# Autodesk Inventor assembly: DarkCeilingSubassembly
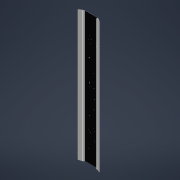
[picture p0: Inventor's stored thumbnail of the model, 180x180]
Saved by Autodesk Inventor 2021 (Build 250183000, 183)
## iProperties
Created: 2021-01-31
Part Number: DarkCeilingSubassembly
Document SubType Name: Assembly
Designer: argon
Author: argon
## Documents named in this file (5)
- C:\Users\argon\OneDrive\Documents\GrabCAD\EngOne Maroons\Ceiling Subassembly\DarkCeilingSubassembly.iam
- C:\Users\argon\OneDrive\Documents\GrabCAD\EngOne Maroons\Ceiling Subassembly\CeilingPanel.ipt
- C:\Users\argon\OneDrive\Documents\GrabCAD\EngOne Maroons\Ceiling Subassembly\StarBackdropPanel.ipt
- C:\Users\argon\OneDrive\Documents\GrabCAD\EngOne Maroons\Ceiling Subassembly\DarkSkyPanel.ipt
- C:\Users\argon\OneDrive\Documents\GrabCAD\EngOne Maroons\Ceiling Subassembly\CeilingLight.ipt
## Components (5 placed, 4 different names)
1. CeilingPanel:1 — Mate:1, Flush:1, Mate:2, Mate:4, Mate:5, Flush:3, Mate:6, Flush:4
2. StarBackdropPanel:1 — Mate:1, Flush:1, Mate:2, Mate:3, Flush:2
3. DarkSkyPanel:1 — Mate:3, Mate:4, Flush:2
4. CeilingLight:1 — Mate:5, Flush:3
5. CeilingLight:2 — Mate:6, Flush:4
## Relationships (10: Mate 6, Flush 4)
- Mate:1: CeilingPanel:1 ↔ StarBackdropPanel:1
- Flush:1: CeilingPanel:1 ↔ StarBackdropPanel:1
- Mate:2: CeilingPanel:1 ↔ StarBackdropPanel:1
- Mate:3: StarBackdropPanel:1 ↔ DarkSkyPanel:1
- Mate:4: CeilingPanel:1 ↔ DarkSkyPanel:1
- Flush:2: StarBackdropPanel:1 ↔ DarkSkyPanel:1
- Mate:5: CeilingPanel:1 ↔ CeilingLight:1
- Flush:3: CeilingPanel:1 ↔ CeilingLight:1
- Mate:6: CeilingPanel:1 ↔ CeilingLight:2
- Flush:4: CeilingPanel:1 ↔ CeilingLight:2
